# Autodesk Inventor assembly: Gripper General
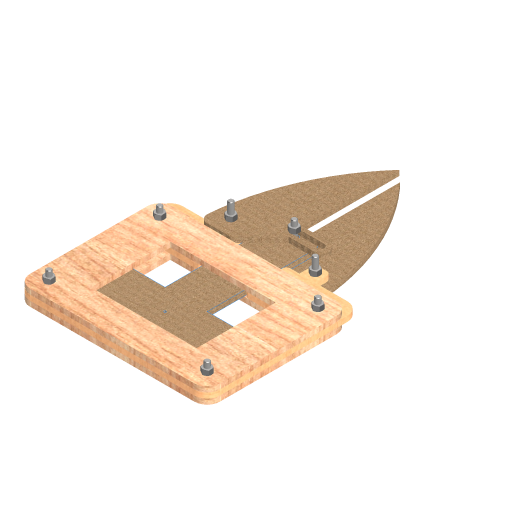
[picture p0: Inventor's stored thumbnail of the model, 512x512]
Saved by Autodesk Inventor 2023.2 (Build 272271000, 271)
## iProperties
Created: 2022-11-11
Part Number: Gripper General
Document SubType Name: Assembly
Designer: Daniel Peña
Author: Daniel Peña
## Documents named in this file (8)
- E:\Daniel DiscoA\Documents\UNAL\ProyectoRobotica\CAD\V3 - BigChungus\Gripper General.iam
- E:\Daniel DiscoA\Documents\UNAL\ProyectoRobotica\CAD\V3 - BigChungus\MarcoBC.ipt
- E:\Daniel DiscoA\Documents\UNAL\ProyectoRobotica\CAD\V3 - BigChungus\PistonBC.ipt
- E:\Daniel DiscoA\Documents\UNAL\ProyectoRobotica\CAD\V3 - BigChungus\Dedo-BC.ipt
- E:\Daniel DiscoA\Documents\UNAL\ProyectoRobotica\CAD\V3 - BigChungus\TapaBC.ipt
- E:\Daniel DiscoA\Documents\UNAL\ProyectoRobotica\CAD\PortaHerramienta\Ventosa.ipt
- E:\Daniel DiscoA\Documents\Inventor\Content Center Files\R2023\en-US\AS 1420\AS 1420 - 1973 - M5 x 25.ipt
- E:\Daniel DiscoA\Documents\Inventor\Content Center Files\R2023\en-US\AS 1112 (2)\AS 1112 - M5  Type 5.ipt
## Components (21 placed, 7 different names)
1. MarcoBC:1 — Slider:1, Rotational:1, Rotational:2, Insert:1, Insert:2, Insert:3, Insert:4, Insert:5, Insert:6, Insert:7, Insert:8, Insert:15, Insert:20
2. PistonBC:1 — Slider:1, Tangent:1, Tangent:2, Mate:2
3. Dedo-BC:1 — Rotational:2, Tangent:1, Insert:21, Mate:4
4. Dedo-BC:2 — Rotational:1, Tangent:2, Insert:13, Mate:3
5. TapaBC:1 — Insert:5, Insert:6, Insert:7, Insert:8, Insert:16, Insert:17, Insert:18, Insert:19
6. Ventosa:1
7. TapaBC:2 — Insert:1, Insert:2, Insert:3, Insert:4, Insert:9, Insert:10, Insert:11, Insert:12
8. AS 1420 - Metric M5 x 25:1 — Insert:9
9. AS 1420 - Metric M5 x 25:2 — Insert:10
10. AS 1420 - Metric M5 x 25:3 — Insert:12
11. AS 1420 - Metric M5 x 25:4 — Insert:11
12. AS 1420 - Metric M5 x 25:5 — Mate:1, Mate:2, Mate:3
13. AS 1420 - Metric M5 x 25:6 — Insert:13
14. AS 1420 - Metric M5 x 25:7 — Insert:15
15. AS 1112 (2) - Metric M5  Type 5:1 — Insert:16
16. AS 1112 (2) - Metric M5  Type 5:2 — Insert:17
17. AS 1112 (2) - Metric M5  Type 5:3 — Insert:18
18. AS 1112 (2) - Metric M5  Type 5:4 — Insert:19
19. AS 1112 (2) - Metric M5  Type 5:5 — Insert:20
20. AS 1112 (2) - Metric M5  Type 5:6 — Insert:21
21. AS 1112 (2) - Metric M5  Type 5:7 — Mate:1, Mate:4
## Relationships (29: Insert 20, Mate 4, RevoluteJoint 2, Tangent 2, TranslationJoint 1)
- Slider:1 [TranslationJoint]: MarcoBC:1 ↔ PistonBC:1
- Rotational:1 [RevoluteJoint]: MarcoBC:1 ↔ Dedo-BC:2
- Rotational:2 [RevoluteJoint]: MarcoBC:1 ↔ Dedo-BC:1
- Tangent:1: PistonBC:1 ↔ Dedo-BC:1
- Tangent:2: PistonBC:1 ↔ Dedo-BC:2
- Insert:1: MarcoBC:1 ↔ TapaBC:2
- Insert:2: MarcoBC:1 ↔ TapaBC:2
- Insert:3: MarcoBC:1 ↔ TapaBC:2
- Insert:4: MarcoBC:1 ↔ TapaBC:2
- Insert:5: MarcoBC:1 ↔ TapaBC:1
- Insert:6: MarcoBC:1 ↔ TapaBC:1
- Insert:7: MarcoBC:1 ↔ TapaBC:1
- Insert:8: MarcoBC:1 ↔ TapaBC:1
- Insert:9: TapaBC:2 ↔ AS 1420 - Metric M5 x 25:1
- Insert:10: TapaBC:2 ↔ AS 1420 - Metric M5 x 25:2
- Insert:11: TapaBC:2 ↔ AS 1420 - Metric M5 x 25:4
- Insert:12: TapaBC:2 ↔ AS 1420 - Metric M5 x 25:3
- Insert:13: Dedo-BC:2 ↔ AS 1420 - Metric M5 x 25:6
- Insert:15: MarcoBC:1 ↔ AS 1420 - Metric M5 x 25:7
- Insert:16: TapaBC:1 ↔ AS 1112 (2) - Metric M5  Type 5:1
- Insert:17: TapaBC:1 ↔ AS 1112 (2) - Metric M5  Type 5:2
- Insert:18: TapaBC:1 ↔ AS 1112 (2) - Metric M5  Type 5:3
- Insert:19: TapaBC:1 ↔ AS 1112 (2) - Metric M5  Type 5:4
- Insert:20: MarcoBC:1 ↔ AS 1112 (2) - Metric M5  Type 5:5
- Insert:21: Dedo-BC:1 ↔ AS 1112 (2) - Metric M5  Type 5:6
- Mate:1: AS 1420 - Metric M5 x 25:5 ↔ AS 1112 (2) - Metric M5  Type 5:7
- Mate:2: PistonBC:1 ↔ AS 1420 - Metric M5 x 25:5
- Mate:3: Dedo-BC:2 ↔ AS 1420 - Metric M5 x 25:5
- Mate:4: Dedo-BC:1 ↔ AS 1112 (2) - Metric M5  Type 5:7
